# Autodesk Inventor assembly: test_assembly
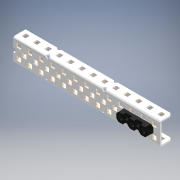
[picture p0: Inventor's stored thumbnail of the model, 180x180]
Saved by Autodesk Inventor 2022 (Build 260153000, 153)
## iProperties
Created: 2021-05-17
Part Number: test_assembly
Document SubType Name: Assembly
Designer: carlo
Author: carlo
## Documents named in this file (3)
- C:\the7dorks.github.io\test_assembly.iam
- C:\the7dorks.github.io\Library 1.2\Structure\C-Channels\Aluminum 1x2x1\1x2x1x13 Aluminum.ipt
- C:\the7dorks.github.io\Library 1.2\Motion\Bearing Flat.ipt
## Components (2 placed, 2 different names)
1. 1x2x1x13 Aluminum:1 — Insert:1, Insert:2
2. Bearing Flat:1 — Insert:1, Insert:2
## Relationships (2: Insert 2)
- Insert:1: 1x2x1x13 Aluminum:1 ↔ Bearing Flat:1
- Insert:2: 1x2x1x13 Aluminum:1 ↔ Bearing Flat:1
